# Autodesk Inventor assembly: box
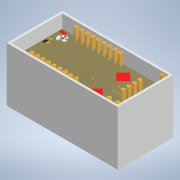
[picture p0: Inventor's stored thumbnail of the model, 180x180]
Saved by Autodesk Inventor 2021 (Build 250183000, 183)
## iProperties
Created: 2021-03-15
Part Number: box
Document SubType Name: Assembly
Designer: kanyk
Author: kanyk
## Documents named in this file (4)
- D:\Project\AllTaskFromTUL\TUL\20202021\ZKO\box.iam
- D:\Project\AllTaskFromTUL\TUL\20202021\ZKO\bottom.ipt
- D:\Project\AllTaskFromTUL\TUL\20202021\ZKO\top.ipt
- D:\Project\AllTaskFromTUL\TUL\20202021\ZKO\LOGIC_LEVEL_CONVERTOR_v3.iam
## Components (3 placed, 3 different names)
1. bottom:1 — Stejný směr:1, Proti sobě:1, Proti sobě:2
2. top:1 — Stejný směr:1
3. LOGIC_LEVEL_CONVERTOR_v3:1 [sub-assembly] — Proti sobě:1, Proti sobě:2
## Relationships (3: Mate 2, Flush 1)
- Stejný směr:1 [Flush]: bottom:1 ↔ top:1
- Proti sobě:1 [Mate]: bottom:1 ↔ LOGIC_LEVEL_CONVERTOR_v3:1
- Proti sobě:2 [Mate]: bottom:1 ↔ LOGIC_LEVEL_CONVERTOR_v3:1
